# Autodesk Inventor assembly: Montagem1
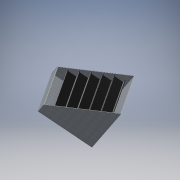
[picture p0: Inventor's stored thumbnail of the model, 180x180]
Saved by Autodesk Inventor 2019.4 (Build 234330000, 330)
## iProperties
Created: 2020-04-10
Part Number: Montagem1
Material: Genérico
Document SubType Name: Assembly
Designer: lucas
Author: lucas
## Documents named in this file (5)
- C:\Users\lucas\source\repos\FrancisTurbine\desenhos\Montagem1.iam
- C:\Users\lucas\source\repos\FrancisTurbine\desenhos\caixa.ipt
- C:\Users\lucas\source\repos\FrancisTurbine\desenhos\tampa.ipt
- C:\Users\lucas\source\repos\FrancisTurbine\desenhos\calha.ipt
- C:\Users\lucas\source\repos\FrancisTurbine\desenhos\trocador1.ipt
## Components (8 placed, 4 different names)
1. caixa:1 — Coincidência:2, Coincidência:3, Alinhamento:2, Coincidência:4, Alinhamento:3, Coincidência:5, Coincidência:6, Alinhamento:4, Coincidência:7, Coincidência:8, Coincidência:9, Coincidência:10, Coincidência:11, Coincidência:12, Coincidência:13, Coincidência:14, Coincidência:15, Coincidência:16, Coincidência:17, Coincidência:18, Coincidência:19, Coincidência:20, Coincidência:21, Coincidência:22
2. tampa:1 — Alinhamento:3, Coincidência:5, Coincidência:6, Alinhamento:4
3. calha:1 — Coincidência:2, Coincidência:3, Alinhamento:2, Coincidência:4
4. trocador1:1 — Coincidência:7, Coincidência:8, Coincidência:9, Coincidência:10
5. trocador1:2 — Coincidência:14, Coincidência:15, Coincidência:16
6. trocador1:3 — Coincidência:11, Coincidência:12, Coincidência:13
7. trocador1:4 — Coincidência:20, Coincidência:21, Coincidência:22
8. trocador1:5 — Coincidência:17, Coincidência:18, Coincidência:19
## Relationships (24: Mate 21, Flush 3)
- Coincidência:2 [Mate]: caixa:1 ↔ calha:1
- Coincidência:3 [Mate]: caixa:1 ↔ calha:1
- Alinhamento:2 [Flush]: caixa:1 ↔ calha:1
- Coincidência:4 [Mate]: caixa:1 ↔ calha:1
- Alinhamento:3 [Flush]: caixa:1 ↔ tampa:1
- Coincidência:5 [Mate]: caixa:1 ↔ tampa:1
- Coincidência:6 [Mate]: caixa:1 ↔ tampa:1
- Alinhamento:4 [Flush]: caixa:1 ↔ tampa:1
- Coincidência:7 [Mate]: caixa:1 ↔ trocador1:1
- Coincidência:8 [Mate]: caixa:1 ↔ trocador1:1
- Coincidência:9 [Mate]: caixa:1 ↔ trocador1:1
- Coincidência:10 [Mate]: caixa:1 ↔ trocador1:1
- Coincidência:11 [Mate]: caixa:1 ↔ trocador1:3
- Coincidência:12 [Mate]: caixa:1 ↔ trocador1:3
- Coincidência:13 [Mate]: caixa:1 ↔ trocador1:3
- Coincidência:14 [Mate]: caixa:1 ↔ trocador1:2
- Coincidência:15 [Mate]: caixa:1 ↔ trocador1:2
- Coincidência:16 [Mate]: caixa:1 ↔ trocador1:2
- Coincidência:17 [Mate]: caixa:1 ↔ trocador1:5
- Coincidência:18 [Mate]: caixa:1 ↔ trocador1:5
- Coincidência:19 [Mate]: caixa:1 ↔ trocador1:5
- Coincidência:20 [Mate]: caixa:1 ↔ trocador1:4
- Coincidência:21 [Mate]: caixa:1 ↔ trocador1:4
- Coincidência:22 [Mate]: caixa:1 ↔ trocador1:4
